# Autodesk Inventor assembly: Assembly1
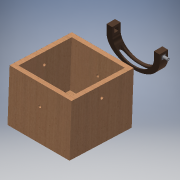
[picture p0: Inventor's stored thumbnail of the model, 180x180]
Saved by Autodesk Inventor 2017 (Build 210142000, 142)
## iProperties
Created: 2017-01-26
Part Number: Assembly1
Document SubType Name: Assembly
Designer: aribu
Author: aribu
## Documents named in this file (4)
- C:\Users\aribu\Dropbox\Kettering\CE-490 CE Capstone\3D Files\Assembly1.iam
- C:\Users\aribu\Dropbox\Kettering\CE-490 CE Capstone\3D Files\Box.ipt
- C:\Users\aribu\Dropbox\Kettering\CE-490 CE Capstone\3D Files\Arms1.ipt
- C:\Users\aribu\Dropbox\Kettering\CE-490 CE Capstone\3D Files\Motor Connection.ipt
## Components (4 placed, 3 different names)
1. Box:1 — Rotational:1, Rotational:2
2. Arms1:1 — Rotational:1
3. Arms1:2 — Rotational:2, Flush:1, Mate:1, Mate:2
4. Motor Connection:1 — Flush:1, Mate:1, Mate:2
## Relationships (5: RevoluteJoint 2, Mate 2, Flush 1)
- Rotational:1 [RevoluteJoint]: Box:1 ↔ Arms1:1
- Rotational:2 [RevoluteJoint]: Box:1 ↔ Arms1:2
- Flush:1: Arms1:2 ↔ Motor Connection:1
- Mate:1: Arms1:2 ↔ Motor Connection:1
- Mate:2: Arms1:2 ↔ Motor Connection:1
